# Autodesk Inventor assembly: Workbench
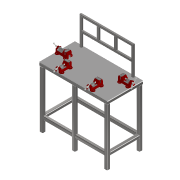
[picture p0: Inventor's stored thumbnail of the model, 180x180]
Saved by Autodesk Inventor 2022 (Build 260148000, 148)
## iProperties
Created: 2021-03-15
Part Number: Workbench
Document SubType Name: Assembly
Designer: jmacmillan
Author: jmacmillan
## Documents named in this file (3)
- C:\Autodesk Inventor 2022 Advanced Assembly Modeling Practice Files\Substitute Model State\Workbench.iam
- C:\Autodesk Inventor 2022 Advanced Assembly Modeling Practice Files\Substitute Model State\Workbench_Frame.iam
- C:\Autodesk Inventor 2022 Advanced Assembly Modeling Practice Files\Substitute Model State\ViseASM.iam
## Components (5 placed, 2 different names)
1. Workbench_Frame:1 [sub-assembly] — Mate:1, Mate:2, Mate:3, Flush:1, Flush:2, Flush:3, Flush:4, Flush:5, Flush:6, Mate:4, Flush:7, Flush:8
2. ViseASM:1 [sub-assembly] — Mate:1, Flush:1, Flush:2
3. ViseASM:2 [sub-assembly] — Mate:3, Flush:3, Flush:5
4. ViseASM:3 [sub-assembly] — Mate:2, Flush:4, Flush:6
5. ViseASM:4 [sub-assembly] — Mate:4, Flush:7, Flush:8
## Relationships (12: Flush 8, Mate 4)
- Mate:1: Workbench_Frame:1 ↔ ViseASM:1
- Mate:2: Workbench_Frame:1 ↔ ViseASM:3
- Mate:3: Workbench_Frame:1 ↔ ViseASM:2
- Flush:1: Workbench_Frame:1 ↔ ViseASM:1
- Flush:2 (-350 mm): Workbench_Frame:1 ↔ ViseASM:1
- Flush:3: Workbench_Frame:1 ↔ ViseASM:2
- Flush:4: Workbench_Frame:1 ↔ ViseASM:3
- Flush:5 (-250 mm): Workbench_Frame:1 ↔ ViseASM:2
- Flush:6 (-250 mm): Workbench_Frame:1 ↔ ViseASM:3
- Mate:4: Workbench_Frame:1 ↔ ViseASM:4
- Flush:7: Workbench_Frame:1 ↔ ViseASM:4
- Flush:8 (-250 mm): Workbench_Frame:1 ↔ ViseASM:4
